# Autodesk Inventor assembly: XWheel
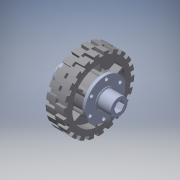
[picture p0: Inventor's stored thumbnail of the model, 180x180]
Saved by Autodesk Inventor 2016 (Build 200138000, 138)
## iProperties
Created: 2016-01-28
Part Number: XWheel
Document SubType Name: Assembly
Designer: 17swamipr
Author: 17swamipr
## Documents named in this file (3)
- C:\Users\17swamipr\Desktop\Robot Assembly 1-27-15 v3.0 Swami\Robot Assembly\Special Assemblies\XWheel.iam
- C:\Users\17swamipr\Desktop\Robot Assembly 1-27-15 v3.0 Swami\Robot Assembly\Special Assemblies\4 in HiGrip Wheel.ipt
- C:\Users\17swamipr\Desktop\Robot Assembly 1-27-15 v3.0 Swami\Robot Assembly\Special Assemblies\am-0096a+500+Hex+Hub+r2.ipt
## Components (3 placed, 2 different names)
1. 4 in HiGrip Wheel:1 — Insert:1, Insert:2, Mate:1, Mate:2, Flush:1
2. am-0096a+500+Hex+Hub+r2:1 — Insert:1, Mate:2
3. am-0096a+500+Hex+Hub+r2:2 — Insert:2, Mate:1
## Relationships (5: Insert 2, Mate 2, Flush 1)
- Insert:1: 4 in HiGrip Wheel:1 ↔ am-0096a+500+Hex+Hub+r2:1
- Insert:2: 4 in HiGrip Wheel:1 ↔ am-0096a+500+Hex+Hub+r2:2
- Mate:1: 4 in HiGrip Wheel:1 ↔ am-0096a+500+Hex+Hub+r2:2
- Mate:2: 4 in HiGrip Wheel:1 ↔ am-0096a+500+Hex+Hub+r2:1
- Flush:1 (53.34 mm): 4 in HiGrip Wheel:1
